# Autodesk Inventor assembly: triangle_brace
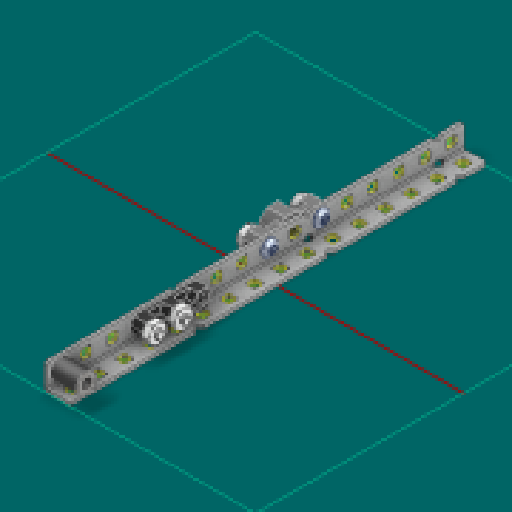
[picture p0: Inventor's stored thumbnail of the model, 512x512]
Saved by Autodesk Inventor 2025 (Build 290162000, 162)
## iProperties
Created: 2024-10-13
Part Number: triangle_brace
Document SubType Name: Assembly
Designer: Averey Ku
Author: Averey Ku
## Documents named in this file (12)
- C:\Users\avere\vex_robotics_high_stakes\hardware\cad\bots\high_stakes_v2\tower\structure\triangle_brace.iam
- C:\Users\avere\vex_robotics_high_stakes\hardware\cad\robpros_cad_lib\Structure\Angle\Aluminum 1x1\Alu Angle 1x1x16.ipt
- C:\Users\avere\vex_robotics_high_stakes\hardware\cad\robpros_cad_lib\Motion\Shaft HS\HS Bearing Flat.ipt
- C:\Users\avere\vex_robotics_high_stakes\hardware\cad\robpros_cad_lib\Motion\Spacers\Spacer Nylon .375 OD\NSpacer .375 OD x .500.ipt
- D:\vex_robotics_high_stakes\hardware\cad\robpros_cad_lib\Motion\Spacers\Spacer Nylon .375 OD.ipt
- C:\Users\avere\vex_robotics_high_stakes\hardware\cad\robpros_cad_lib\Motion\Spacers\Washer Steel\SWasher .375 OD x .015625.ipt
- D:\vex_robotics_high_stakes\hardware\cad\robpros_cad_lib\Motion\Spacers\Washer Steel.ipt
- C:\Users\avere\vex_robotics_high_stakes\hardware\cad\VEX-CAD-Inventor\Structure\Hardware\Screw Shoulder Robosource\SScrew Shoulder Smooth .500 x .04.ipt
- D:\vex_robotics_high_stakes\hardware\cad\VEX-CAD-Inventor\Structure\Hardware\Screw Shoulder Robosource.ipt
- C:\Users\avere\vex_robotics_high_stakes\hardware\cad\VEX-CAD-Inventor\Structure\Hardware\Nut Nylon\Nut Nylon - White.ipt
- D:\vex_robotics_high_stakes\hardware\cad\VEX-CAD-Inventor\Structure\Hardware\Nut Nylon.ipt
- C:\Users\avere\vex_robotics_high_stakes\hardware\cad\robpros_cad_lib\Quick Assemblies\bearing_flat_w_hardware_offset.iam
## Components (9 placed, 7 different names)
1. Alu Angle 1x1x16:1 — Mate:2, Angle:1, Mate:3, Flush:1, Insert:4, Insert:5, Insert:7, Insert:9, Mate:7
2. HS Bearing Flat:1 — Insert:6, Insert:8
3. NSpacer .375 OD x .500:1 — Insert:3, Insert:4
4. SWasher .375 OD x .015625:1 — Insert:3
5. SScrew Shoulder Smooth .500 x .04:1 — Insert:5
6. Nut Nylon - White:1 — Insert:6
7. SScrew Shoulder Smooth .500 x .04:2 — Insert:7
8. Nut Nylon - White:2 — Insert:8
9. bearing_flat_w_hardware_offset:1 [sub-assembly] — Insert:9, Mate:7
## Relationships (16: Insert 8, Mate 6, Angle 1, Flush 1)
- [Insert]: Alu Angle 1x1x16:1 ↔ HS Bearing Flat:1
- [Mate]: Alu Angle 1x1x16:1 ↔ HS Bearing Flat:1
- Mate:2 (6.35 mm): Alu Angle 1x1x16:1
- Angle:1 (0 deg): Alu Angle 1x1x16:1
- Mate:3: Alu Angle 1x1x16:1
- Flush:1: Alu Angle 1x1x16:1
- Insert:3: NSpacer .375 OD x .500:1 ↔ SWasher .375 OD x .015625:1
- Insert:4: Alu Angle 1x1x16:1 ↔ NSpacer .375 OD x .500:1
- [Mate]: SScrew Shoulder Smooth .500 x .04:1 ↔ Nut Nylon - White:1
- Insert:5: Alu Angle 1x1x16:1 ↔ SScrew Shoulder Smooth .500 x .04:1
- Insert:6: HS Bearing Flat:1 ↔ Nut Nylon - White:1
- [Mate]: SScrew Shoulder Smooth .500 x .04:2 ↔ Nut Nylon - White:2
- Insert:7: Alu Angle 1x1x16:1 ↔ SScrew Shoulder Smooth .500 x .04:2
- Insert:8: HS Bearing Flat:1 ↔ Nut Nylon - White:2
- Insert:9: Alu Angle 1x1x16:1 ↔ bearing_flat_w_hardware_offset:1
- Mate:7: Alu Angle 1x1x16:1 ↔ bearing_flat_w_hardware_offset:1
## Named parameters: d12_d3 = 0 mm, d15_d12_d3 = 0 mm
